# Autodesk Inventor assembly: M12_BNC
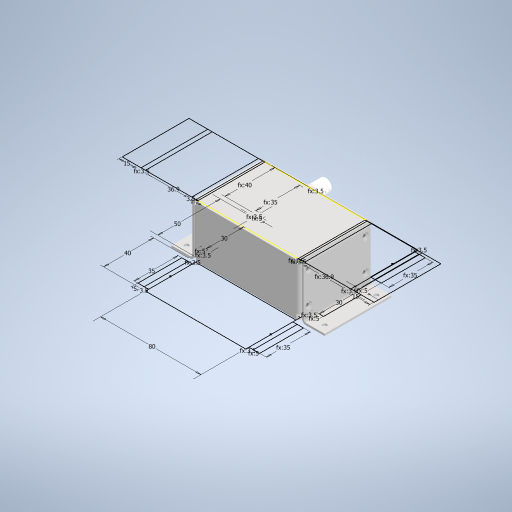
[picture p0: Inventor's stored thumbnail of the model, 512x512]
Saved by Autodesk Inventor 2024 (Build 280153000, 153)
## iProperties
Created: 2025-10-28
Part Number: M12_BNC
Document SubType Name: Assembly
Designer: alexi
Author: alexi
## Documents named in this file (4)
- C:\Jeonghyun\SNU_GIT\QSTL_M12C_BNC\Enclosure\M12_BNC.iam
- C:\Jeonghyun\SNU_GIT\QSTL_M12C_BNC\Enclosure\Bottom.ipt
- C:\Jeonghyun\SNU_GIT\QSTL_M12C_BNC\Enclosure\QSTL_M12C_BNC\QSTL_M12C_BNC.iam
- C:\Jeonghyun\SNU_GIT\QSTL_M12C_BNC\Enclosure\Top.ipt
## Components (3 placed, 3 different names)
1. Bottom:1 — 플러쉬:1, 플러쉬:2
2. QSTL_M12C_BNC:1 [sub-assembly]
3. Top:1 — 플러쉬:1, 플러쉬:2
## Relationships (2: Flush 2)
- 플러쉬:1 [Flush]: Bottom:1 ↔ Top:1
- 플러쉬:2 [Flush]: Bottom:1 ↔ Top:1
